# Autodesk Inventor assembly: Battery_Pack
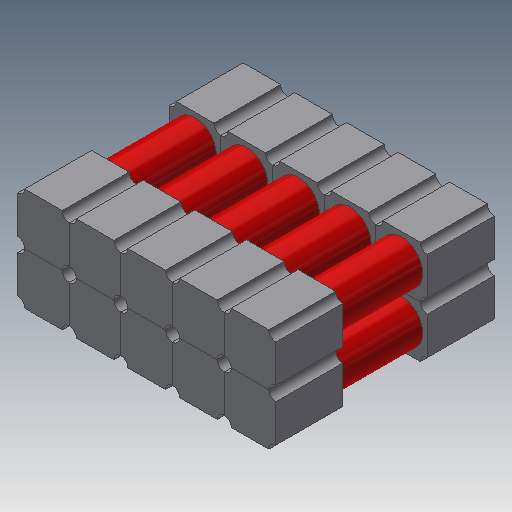
[picture p0: Inventor's stored thumbnail of the model, 512x512]
Saved by Autodesk Inventor 2018 (Build 220112000, 112)
## iProperties
Created: 2019-09-04
Part Number: Battery_Pack
Document SubType Name: Assembly
Designer: Clevo
Author: Clevo
## Documents named in this file (2)
- E:\Hardware_Accelerated_Robot\Hardware\Battery\Battery_Pack.iam
- E:\Hardware_Accelerated_Robot\Hardware\Battery\Battery_Module.iam
## Components (10 placed, 1 different names)
1. Battery_Module:1 [sub-assembly] — Mate:1, Flush:1, Flush:2, Mate:2, Flush:3, Flush:4, Mate:9, Flush:17
2. Battery_Module:2 [sub-assembly] — Mate:1, Flush:1, Flush:2, Mate:4, Flush:7, Flush:8
3. Battery_Module:3 [sub-assembly] — Mate:2, Flush:3, Flush:4, Mate:3, Flush:5, Flush:6
4. Battery_Module:4 [sub-assembly] — Mate:3, Flush:5, Flush:6
5. Battery_Module:5 [sub-assembly] — Mate:4, Flush:7, Flush:8, Flush:18
6. Battery_Module:6 [sub-assembly] — Mate:9, Flush:17
7. Battery_Module:7 [sub-assembly]
8. Battery_Module:8 [sub-assembly]
9. Battery_Module:9 [sub-assembly]
10. Battery_Module:10 [sub-assembly] — Flush:18
## Relationships (27: Flush 18, Mate 9)
- Mate:1: Battery_Module:1 ↔ Battery_Module:2
- Flush:1: Battery_Module:1 ↔ Battery_Module:2
- Flush:2: Battery_Module:1 ↔ Battery_Module:2
- Mate:2: Battery_Module:1 ↔ Battery_Module:3
- Flush:3: Battery_Module:1 ↔ Battery_Module:3
- Flush:4: Battery_Module:1 ↔ Battery_Module:3
- Mate:3: Battery_Module:3 ↔ Battery_Module:4
- Flush:5: Battery_Module:3 ↔ Battery_Module:4
- Flush:6: Battery_Module:3 ↔ Battery_Module:4
- Mate:4: Battery_Module:2 ↔ Battery_Module:5
- Flush:7: Battery_Module:2 ↔ Battery_Module:5
- Flush:8: Battery_Module:2 ↔ Battery_Module:5
- [Mate]: Battery_Module:6 ↔ Battery_Module:7
- [Flush]: Battery_Module:6 ↔ Battery_Module:7
- [Flush]: Battery_Module:6 ↔ Battery_Module:7
- [Mate]: Battery_Module:6 ↔ Battery_Module:8
- [Flush]: Battery_Module:6 ↔ Battery_Module:8
- [Flush]: Battery_Module:6 ↔ Battery_Module:8
- [Mate]: Battery_Module:8 ↔ Battery_Module:9
- [Flush]: Battery_Module:8 ↔ Battery_Module:9
- [Flush]: Battery_Module:8 ↔ Battery_Module:9
- [Mate]: Battery_Module:7 ↔ Battery_Module:10
- [Flush]: Battery_Module:7 ↔ Battery_Module:10
- [Flush]: Battery_Module:7 ↔ Battery_Module:10
- Mate:9: Battery_Module:1 ↔ Battery_Module:6
- Flush:17: Battery_Module:1 ↔ Battery_Module:6
- Flush:18: Battery_Module:5 ↔ Battery_Module:10
## Named parameters: d12_d10 = 0 mm, d13_d11 = 0 mm, d14_d1 = 0 mm, d15_d2 = 0 mm, d16_d3 = 0 mm, d17_d4 = 0 mm, d18_d5 = 0 mm, d19_d6 = 0 mm, d20_d7 = 0 mm, d21_d8 = 0 mm, d22_d9 = 0 mm, d23_d0 = 0 mm
